# Autodesk Inventor assembly: rollers_plate
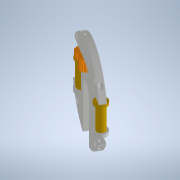
[picture p0: Inventor's stored thumbnail of the model, 180x180]
Saved by Autodesk Inventor 2021 (Build 250183000, 183)
## iProperties
Created: 2024-02-12
Part Number: rollers_plate
Document SubType Name: Assembly
Designer: Sebastián
Author: Sebastián
## Documents named in this file (8)
- C:\Users\Sebastián\Documents\Inventor\PLD SAP\rollers_plate.iam
- C:\Users\Sebastián\Documents\Inventor\PLD SAP\shaft_6mm.ipt
- C:\Users\Sebastián\Documents\Inventor\PLD SAP\placa_rollers\Design Accelerator\Spur Gears1.iam
- C:\Users\Sebastián\Documents\Inventor\PLD SAP\rewwind_roller.ipt
- C:\Users\Sebastián\Documents\Inventor\PLD SAP\unwind_roller.ipt
- C:\Users\Sebastián\Documents\Inventor\PLD SAP\placa_rollers_v2.ipt
- C:\Users\Sebastián\Documents\Inventor\PLD SAP\unwind_roller_adjuster.ipt
- C:\Users\Sebastián\Documents\Inventor\PLD SAP\roller_adjuster.ipt
## Components (8 placed, 7 different names)
1. shaft_6mm:1 — Mate:1, Cylindrical:1, Cylindrical:2
2. shaft_6mm:2 — Mate:3, Cylindrical:3
3. Spur Gears:1 [sub-assembly] — Mate:1, Mate:3, Mate:4, Mate:6
4. rewwind_roller:1 — Cylindrical:1, Mate:4, Mate:5, Rotational:3
5. unwind_roller:1 — Rotational:1, Rotational:2
6. placa_rollers_v2:1 — Rotational:1, Cylindrical:2, Mate:5, Cylindrical:3, Mate:6
7. unwind_roller_adjuster:1 — Rotational:2
8. roller_adjuster:1 — Rotational:3
## Relationships (11: Mate 5, RevoluteJoint 3, CylindricalJoint 3)
- Mate:1: shaft_6mm:1 ↔ Spur Gears:1
- Mate:3: shaft_6mm:2 ↔ Spur Gears:1
- Rotational:1 [RevoluteJoint]: unwind_roller:1 ↔ placa_rollers_v2:1
- Cylindrical:1: shaft_6mm:1 ↔ rewwind_roller:1
- Mate:4: Spur Gears:1 ↔ rewwind_roller:1
- Cylindrical:2: shaft_6mm:1 ↔ placa_rollers_v2:1
- Mate:5: rewwind_roller:1 ↔ placa_rollers_v2:1
- Cylindrical:3: shaft_6mm:2 ↔ placa_rollers_v2:1
- Mate:6: Spur Gears:1 ↔ placa_rollers_v2:1
- Rotational:2 [RevoluteJoint]: unwind_roller:1 ↔ unwind_roller_adjuster:1
- Rotational:3 [RevoluteJoint]: rewwind_roller:1 ↔ roller_adjuster:1
